# Autodesk Inventor assembly: 車輪取り付け部
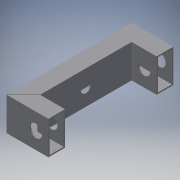
[picture p0: Inventor's stored thumbnail of the model, 180x180]
Saved by Autodesk Inventor 2018 (Build 220112000, 112)
## iProperties
Created: 2017-09-10
Part Number: 車輪取り付け部
Material: 一般
Document SubType Name: Assembly
Designer: mura5
Author: mura5
## Documents named in this file (3)
- C:\Users\mura5\Documents\RBBR\cart\車輪取り付け部.iam
- C:\Users\mura5\Documents\RBBR\cart\Pipe3.ipt
- C:\Users\mura5\Documents\RBBR\cart\Pipe4.ipt
## Components (3 placed, 2 different names)
1. Pipe3:1 — リジッド:1, リジッド:2
2. Pipe4:1 — リジッド:1
3. Pipe4:2 — リジッド:2
## Relationships (2: WeldJoint 2)
- リジッド:1 [WeldJoint]: Pipe3:1 ↔ Pipe4:1
- リジッド:2 [WeldJoint]: Pipe3:1 ↔ Pipe4:2
